# Autodesk Inventor assembly: dining_table
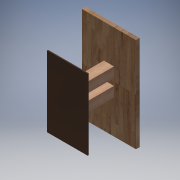
[picture p0: Inventor's stored thumbnail of the model, 180x180]
Saved by Autodesk Inventor 2019 (Build 230136000, 136)
## iProperties
Created: 2019-04-29
Part Number: dining_table
Document SubType Name: Assembly
Designer: Alex
Author: Alex
## Documents named in this file (4)
- P:\Alex\Git\3d_models\dining_table\dining_table.iam
- P:\Alex\Git\3d_models\dining_table\adapter.ipt
- P:\Alex\Git\3d_models\dining_table\stand.ipt
- P:\Alex\Git\3d_models\dining_table\tabletop.ipt
## Components (5 placed, 3 different names)
1. adapter:1 — Mate:3, Flush:3, Mate:5, Flush:4
2. stand:1 — Mate:3, Flush:6, Flush:8, Mate:7
3. tabletop:1 — Flush:3, Flush:4, Flush:5, Flush:6, Flush:7, Flush:8, Mate:6, Flush:9, Flush:10
4. stand:2 — Mate:5, Flush:5, Flush:7
5. tabletop:2 — Mate:6, Flush:9, Flush:10, Mate:7
## Relationships (12: Flush 8, Mate 4)
- Mate:3: adapter:1 ↔ stand:1
- Flush:3 (-175 mm): adapter:1 ↔ tabletop:1
- Mate:5: adapter:1 ↔ stand:2
- Flush:4 (100 mm): adapter:1 ↔ tabletop:1
- Flush:5 (-500 mm): tabletop:1 ↔ stand:2
- Flush:6 (-500 mm): stand:1 ↔ tabletop:1
- Flush:7 (325 mm): tabletop:1 ↔ stand:2
- Flush:8 (325 mm): stand:1 ↔ tabletop:1
- Mate:6: tabletop:1 ↔ tabletop:2
- Flush:9: tabletop:1 ↔ tabletop:2
- Flush:10: tabletop:1 ↔ tabletop:2
- Mate:7: stand:1 ↔ tabletop:2
